# Autodesk Inventor assembly: montagem_planta
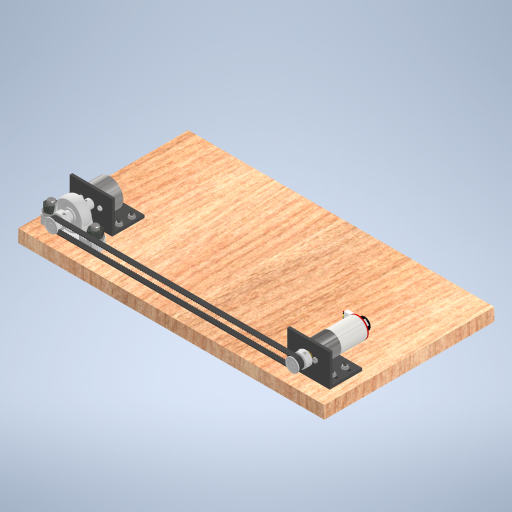
[picture p0: Inventor's stored thumbnail of the model, 512x512]
Saved by Autodesk Inventor 2023 (Build 270158000, 158)
## iProperties
Created: 2022-10-11
Part Number: montagem_planta
Document SubType Name: Assembly
Designer: klebe
Author: klebe
## Documents named in this file (23)
- C:\Users\klebe\OneDrive\Documents\GitHub\Eng_Meca\6º período\Lab_Analise\esteira\montagem_planta.iam
- C:\Users\klebe\OneDrive\Documents\GitHub\Eng_Meca\6º período\Lab_Analise\esteira\Base\base1.ipt
- C:\Users\klebe\OneDrive\Documents\GitHub\Eng_Meca\6º período\Lab_Analise\esteira\motor\JGA25-371_12VDC_85RPM.ipt
- C:\Users\klebe\OneDrive\Documents\GitHub\Eng_Meca\6º período\Lab_Analise\esteira\suporte\suporte.ipt
- C:\Users\klebe\OneDrive\Documents\GitHub\Eng_Meca\6º período\Lab_Analise\esteira\polia\poliaGT2 20B5.ipt
- C:\Users\klebe\OneDrive\Documents\GitHub\Eng_Meca\6º período\Lab_Analise\esteira\Acoplador\acoplador.ipt
- C:\Users\klebe\OneDrive\Documents\GitHub\Eng_Meca\6º período\Lab_Analise\esteira\Acoplador\suporte 2.ipt
- C:\Users\klebe\OneDrive\Documents\GitHub\Eng_Meca\6º período\Lab_Analise\esteira\motor\motor_sensor.ipt
- C:\Users\klebe\OneDrive\Documents\GitHub\Eng_Meca\6º período\Lab_Analise\esteira\esteira\correia.ipt
- C:\Users\klebe\OneDrive\Documents\Inventor\Content Center Files\R2023\en-US\ISO 7089\ISO 7089 - 3 - 140 HV(1).ipt
- C:\Users\klebe\OneDrive\Documents\Inventor\Content Center Files\R2023\en-US\ISO 4032(2)\ISO 4032 - M3 - ISO.ipt
- C:\Users\klebe\OneDrive\Documents\Inventor\Content Center Files\R2023\en-US\DIN 84\DIN 84 - M3 x 12.ipt
- C:\Users\klebe\OneDrive\Documents\Inventor\Content Center Files\R2023\en-US\DIN 7985 (H)\DIN 7985 (H) - M2,5x5-H.ipt
- C:\Users\klebe\OneDrive\Documents\Inventor\Content Center Files\R2023\en-US\ISO 7046-1 H(1)\ISO 7046-1 - M3 x 25_ - 4.8 - H - ISO.ipt
- C:\Users\klebe\OneDrive\Documents\GitHub\Eng_Meca\6º período\Lab_Analise\esteira\acoplador sensor.ipt
- C:\Users\klebe\OneDrive\Documents\Inventor\Content Center Files\R2023\en-US\AS 1421(1)\AS 1421 - M3x6 Cone Point.ipt
- C:\Users\klebe\OneDrive\Documents\Inventor\Content Center Files\R2023\en-US\ANSI B18.3.6M(00)\ANSI B18.3.6M - M3x0,5 x 4(4).ipt
- C:\Users\klebe\OneDrive\Documents\GitHub\Eng_Meca\6º período\Lab_Analise\esteira\Mancal\PK000.ipt
- C:\Users\klebe\OneDrive\Documents\GitHub\Eng_Meca\6º período\Lab_Analise\esteira\Mancal\suporte_mancal.ipt
- C:\Users\klebe\OneDrive\Documents\Inventor\Content Center Files\R2023\en-US\ISO 4762(2)\ISO 4762 - M8 x 30ISO.ipt
- C:\Users\klebe\OneDrive\Documents\Inventor\Content Center Files\R2023\en-US\ISO 7089\ISO 7089 - 8 - 140 HV(1).ipt
- C:\Users\klebe\OneDrive\Documents\Inventor\Content Center Files\R2023\en-US\ISO 4033(2)\ISO 4033 - M8 - ISO.ipt
- C:\Users\klebe\OneDrive\Documents\Inventor\Content Center Files\R2023\en-US\AS 1421(1)\AS 1421 - M4x6 Cone Point.ipt
## Components (51 placed, 22 different names)
1. base1:1 — Mate:2, Mate:36, Mate:37, Mate:38, Mate:39, Mate:40, Mate:41, Mate:42, Mate:43, Mate:45, Mate:47, Mate:49, Mate:51, Mate:52, Mate:53, Mate:54, Mate:55, Mate:57, Mate:59, Mate:61, Flush:1, Mate:63, Mate:64, Mate:65, Mate:66, Mate:67, Mate:69
2. correia:1 — Rotational:3, Rotational:9
3. motor — Rigid:8, Rotational:10
4. suporte:1 — Rigid:8, Insert:61, Insert:62, Mate:44, Mate:46, Mate:48, Mate:50
5. acoplador:1 — Rotational:6
6. poliaGT2 20B5:1 — Rotational:3, Rotational:6, Rotational:10
7. motor_sensor:1 — Rigid:6
8. suporte 2:1 — Rigid:6, Mate:2, Insert:59, Insert:60, Rotational:8, Mate:56, Mate:58, Mate:60, Mate:62
9. acoplador sensor:1 — Rotational:7, Rotational:8, Rigid:10, Rotational:11
10. Broached Hexagon Socket Set Screw - Cone Point - Metric M3x0,5 x 4:1 — Rigid:10
11. poliaGT2 20B5:2 — Rotational:7, Rotational:9, Rigid:11, Rigid:14
12. AS 1421 Cone Point - Metric M3x6 Cone Point:1 — Rigid:11
13. AS 1421 Cone Point - Metric M3x6 Cone Point:2 — Rigid:14
14. AS 1421 Cone Point - Metric M4x6 Cone Point:2 — Rigid:13
15. AS 1421 Cone Point - Metric M4x6 Cone Point:1 — Rigid:12
16. ISO 4033 M8:2 — Insert:72
17. ISO 7089 8:2 — Mate:69, Mate:70, Insert:72
18. ISO 4762 M8 x 30:2 — Mate:65, Mate:66
19. ISO 4033 M8:1 — Insert:71
20. ISO 7089 8:1 — Mate:67, Mate:68, Insert:71
21. ISO 4762 M8 x 30:1 — Mate:63, Mate:64
22. suporte_mancal:1 — Flush:1, Rigid:15
23. Mancal PK000 — Rotational:11, Mate:68, Mate:70, Rigid:12, Rigid:13, Rigid:15
24. ISO 7046-1 H M3 x 25 - 4.8 - H:2 — Mate:40
25. ISO 7046-1 H M3 x 25 - 4.8 - H:1 — Mate:39
26. ISO 7046-1 H M3 x 25 - 4.8 - H:3 — Mate:41
27. ISO 7046-1 H M3 x 25 - 4.8 - H:4 — Mate:42
28. ISO 4032 M3:1 — Insert:63
29. ISO 4032 M3:2 — Insert:64
30. ISO 4032 M3:3 — Insert:65
31. ISO 4032 M3:4 — Insert:66
32. ISO 7089 3:1 — Mate:43, Mate:44, Insert:63
33. ISO 7089 3:2 — Mate:45, Mate:46, Insert:64
34. ISO 7089 3:3 — Mate:47, Mate:48, Insert:65
35. ISO 7089 3:4 — Mate:49, Mate:50, Insert:66
36. DIN 84 - replaced by DIN EN ISO 1207 M3 x 12:3 — Insert:61
37. DIN 84 - replaced by DIN EN ISO 1207 M3 x 12:4 — Insert:62
38. ISO 7046-1 H M3 x 25 - 4.8 - H:5 — Mate:51
39. ISO 7089 3:5 — Mate:55, Mate:56, Insert:67
40. ISO 4032 M3:5 — Insert:67
41. ISO 7046-1 H M3 x 25 - 4.8 - H:6 — Mate:52
42. ISO 7046-1 H M3 x 25 - 4.8 - H:7 — Mate:53
43. ISO 7046-1 H M3 x 25 - 4.8 - H:8 — Mate:54
44. ISO 7089 3:6 — Mate:57, Mate:58, Insert:68
45. ISO 7089 3:7 — Mate:59, Mate:60, Insert:69
46. ISO 7089 3:8 — Mate:61, Mate:62, Insert:70
47. ISO 4032 M3:6 — Insert:68
48. ISO 4032 M3:7 — Insert:69
49. ISO 4032 M3:8 — Insert:70
50. DIN 7985 (H) M2,5x5-H:1 — Insert:59
51. DIN 7985 (H) M2,5x5-H:2 — Insert:60
## Relationships (66: Mate 36, Insert 14, WeldJoint 8, RevoluteJoint 7, Flush 1)
- Rigid:6 [WeldJoint]: motor_sensor:1 ↔ suporte 2:1
- Rotational:3 [RevoluteJoint] (0.5 mm): correia:1 ↔ poliaGT2 20B5:1
- Mate:2: base1:1 ↔ suporte 2:1
- Rigid:8 [WeldJoint]: motor ↔ suporte:1
- Mate:36: base1:1
- Mate:37: base1:1
- Rotational:6 [RevoluteJoint]: acoplador:1 ↔ poliaGT2 20B5:1
- Mate:38: base1:1
- Insert:59: suporte 2:1 ↔ DIN 7985 (H) M2,5x5-H:1
- Insert:60: suporte 2:1 ↔ DIN 7985 (H) M2,5x5-H:2
- Insert:61: suporte:1 ↔ DIN 84 - replaced by DIN EN ISO 1207 M3 x 12:3
- Insert:62: suporte:1 ↔ DIN 84 - replaced by DIN EN ISO 1207 M3 x 12:4
- Mate:39: base1:1 ↔ ISO 7046-1 H M3 x 25 - 4.8 - H:1
- Mate:40: base1:1 ↔ ISO 7046-1 H M3 x 25 - 4.8 - H:2
- Mate:41: base1:1 ↔ ISO 7046-1 H M3 x 25 - 4.8 - H:3
- Mate:42: base1:1 ↔ ISO 7046-1 H M3 x 25 - 4.8 - H:4
- Mate:43: base1:1 ↔ ISO 7089 3:1
- Mate:44: suporte:1 ↔ ISO 7089 3:1
- Mate:45: base1:1 ↔ ISO 7089 3:2
- Mate:46: suporte:1 ↔ ISO 7089 3:2
- Mate:47: base1:1 ↔ ISO 7089 3:3
- Mate:48: suporte:1 ↔ ISO 7089 3:3
- Mate:49: base1:1 ↔ ISO 7089 3:4
- Mate:50: suporte:1 ↔ ISO 7089 3:4
- Insert:63: ISO 4032 M3:1 ↔ ISO 7089 3:1
- Insert:64: ISO 4032 M3:2 ↔ ISO 7089 3:2
- Insert:65: ISO 4032 M3:3 ↔ ISO 7089 3:3
- Insert:66: ISO 4032 M3:4 ↔ ISO 7089 3:4
- Rotational:7 [RevoluteJoint]: acoplador sensor:1 ↔ poliaGT2 20B5:2
- Rotational:8 [RevoluteJoint] (-1 mm): suporte 2:1 ↔ acoplador sensor:1
- Rotational:9 [RevoluteJoint] (2 mm): correia:1 ↔ poliaGT2 20B5:2
- Rotational:10 [RevoluteJoint] (-5.5 mm): motor ↔ poliaGT2 20B5:1
- Mate:51: base1:1 ↔ ISO 7046-1 H M3 x 25 - 4.8 - H:5
- Mate:52: base1:1 ↔ ISO 7046-1 H M3 x 25 - 4.8 - H:6
- Mate:53: base1:1 ↔ ISO 7046-1 H M3 x 25 - 4.8 - H:7
- Mate:54: base1:1 ↔ ISO 7046-1 H M3 x 25 - 4.8 - H:8
- Mate:55: base1:1 ↔ ISO 7089 3:5
- Mate:56: suporte 2:1 ↔ ISO 7089 3:5
- Mate:57: base1:1 ↔ ISO 7089 3:6
- Mate:58: suporte 2:1 ↔ ISO 7089 3:6
- Mate:59: base1:1 ↔ ISO 7089 3:7
- Mate:60: suporte 2:1 ↔ ISO 7089 3:7
- Mate:61: base1:1 ↔ ISO 7089 3:8
- Mate:62: suporte 2:1 ↔ ISO 7089 3:8
- Insert:67: ISO 7089 3:5 ↔ ISO 4032 M3:5
- Insert:68: ISO 7089 3:6 ↔ ISO 4032 M3:6
- Insert:69: ISO 7089 3:7 ↔ ISO 4032 M3:7
- Insert:70: ISO 7089 3:8 ↔ ISO 4032 M3:8
- Rigid:10 [WeldJoint]: acoplador sensor:1 ↔ Broached Hexagon Socket Set Screw - Cone Point - Metric M3x0,5 x 4:1
- Rigid:11 [WeldJoint]: poliaGT2 20B5:2 ↔ AS 1421 Cone Point - Metric M3x6 Cone Point:1
- Rotational:11 [RevoluteJoint] (10 mm): acoplador sensor:1 ↔ Mancal PK000
- Flush:1: base1:1 ↔ suporte_mancal:1
- Mate:63: base1:1 ↔ ISO 4762 M8 x 30:1
- Mate:64: base1:1 ↔ ISO 4762 M8 x 30:1
- Mate:65: base1:1 ↔ ISO 4762 M8 x 30:2
- Mate:66: base1:1 ↔ ISO 4762 M8 x 30:2
- Mate:67: base1:1 ↔ ISO 7089 8:1
- Mate:68: ISO 7089 8:1 ↔ Mancal PK000
- Mate:69: base1:1 ↔ ISO 7089 8:2
- Mate:70: ISO 7089 8:2 ↔ Mancal PK000
- Insert:71: ISO 4033 M8:1 ↔ ISO 7089 8:1
- Insert:72: ISO 4033 M8:2 ↔ ISO 7089 8:2
- Rigid:12 [WeldJoint]: AS 1421 Cone Point - Metric M4x6 Cone Point:1 ↔ Mancal PK000
- Rigid:13 [WeldJoint]: AS 1421 Cone Point - Metric M4x6 Cone Point:2 ↔ Mancal PK000
- Rigid:14 [WeldJoint]: poliaGT2 20B5:2 ↔ AS 1421 Cone Point - Metric M3x6 Cone Point:2
- Rigid:15 [WeldJoint]: suporte_mancal:1 ↔ Mancal PK000
